# Autodesk Inventor assembly: Tamale - V1
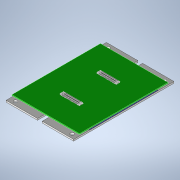
[picture p0: Inventor's stored thumbnail of the model, 180x180]
Saved by Autodesk Inventor 2022 (Build 260153000, 153)
## iProperties
Created: 2022-02-01
Part Number: Tamale - V1
Document SubType Name: Assembly
Designer: Caleb
Author: Caleb
## Documents named in this file (8)
- C:\Users\Caleb\Desktop\nebraska-silicon-lab\Hardware\ETL\modules\tamale\Tamale - V1p2.iam
- C:\Users\Caleb\Desktop\nebraska-silicon-lab\Hardware\ETL\modules\tamale\BBM.iam
- C:\Users\Caleb\Desktop\nebraska-silicon-lab\Hardware\ETL\modules\tamale\Coverplate Film.ipt
- C:\Users\Caleb\Desktop\nebraska-silicon-lab\Hardware\ETL\modules\tamale\Sensor Placement Film.ipt
- C:\Users\Caleb\Desktop\nebraska-silicon-lab\Hardware\ETL\modules\tamale\Mock Module PCB - V2p2.iam
- C:\Users\Caleb\Desktop\nebraska-silicon-lab\Hardware\ETL\modules\tamale\Long Wirebond A.ipt
- C:\Users\Caleb\Desktop\nebraska-silicon-lab\Hardware\ETL\modules\tamale\Long Wirebond B.ipt
- C:\Users\Caleb\Desktop\nebraska-silicon-lab\Hardware\ETL\modules\tamale\Baseplate Extended.ipt
## Components (150 placed, 7 different names)
1. Baseplate Extended:1 — Mate:12, Angle:5, Flush:15
2. BBM:1 [sub-assembly] — Mate:2, Angle:2, Flush:1, Flush:4, Mate:5, Flush:11
3. BBM:2 [sub-assembly] — Mate:3, Angle:1, Flush:2, Flush:4
4. BBM:3 [sub-assembly] — Mate:1, Angle:3, Flush:1, Flush:3, Mate:5, Mate:6, Flush:12
5. BBM:4 [sub-assembly] — Mate:4, Angle:4, Flush:2, Flush:3, Mate:6, Mate:10, Mate:11, Flush:9, Flush:10, Flush:14
6. Mock Module PCB - V2p2:1 [sub-assembly] — Mate:1, Mate:2, Mate:3, Mate:4, Angle:1, Angle:2, Angle:3, Angle:4, Flush:11, Angle:5, Flush:15
7. Coverplate Film:1 — Mate:10, Flush:12, Flush:14, Mate:12
8. Sensor Placement Film:1 — Mate:11, Flush:9, Flush:10
9. Long Wirebond A:1
10. Long Wirebond A:2
11. Long Wirebond A:3
12. Long Wirebond A:4
13. Long Wirebond A:5
14. Long Wirebond A:6
15. Long Wirebond A:7
16. Long Wirebond A:8
17. Long Wirebond A:9
18. Long Wirebond A:10
19. Long Wirebond A:11
20. Long Wirebond A:12
21. Long Wirebond A:13
22. Long Wirebond A:14
23. Long Wirebond A:15
24. Long Wirebond A:16
25. Long Wirebond A:17
26. Long Wirebond A:18
27. Long Wirebond A:19
28. Long Wirebond A:20
29. Long Wirebond A:21
30. Long Wirebond A:22
31. Long Wirebond A:23
32. Long Wirebond A:24
33. Long Wirebond A:25
34. Long Wirebond A:26
35. Long Wirebond A:27
36. Long Wirebond A:28
37. Long Wirebond A:29
38. Long Wirebond A:30
39. Long Wirebond A:31
40. Long Wirebond A:32
41. Long Wirebond A:33
42. Long Wirebond A:34
43. Long Wirebond A:35
44. Long Wirebond A:36
45. Long Wirebond A:37
46. Long Wirebond A:38
47. Long Wirebond A:39
48. Long Wirebond A:40
49. Long Wirebond A:41
50. Long Wirebond A:42
51. Long Wirebond A:43
52. Long Wirebond A:44
53. Long Wirebond A:45
54. Long Wirebond A:46
55. Long Wirebond A:47
56. Long Wirebond A:48
57. Long Wirebond A:49
58. Long Wirebond A:50
59. Long Wirebond A:51
60. Long Wirebond A:52
61. Long Wirebond A:53
62. Long Wirebond A:54
63. Long Wirebond A:55
64. Long Wirebond A:56
65. Long Wirebond A:57
66. Long Wirebond A:58
67. Long Wirebond A:59
68. Long Wirebond A:60
69. Long Wirebond A:61
70. Long Wirebond A:62
71. Long Wirebond A:63
72. Long Wirebond A:64
73. Long Wirebond A:65
74. Long Wirebond A:66
75. Long Wirebond A:67
76. Long Wirebond A:68
77. Long Wirebond A:69
78. Long Wirebond A:70
79. Long Wirebond A:71
80. Long Wirebond B:1
81. Long Wirebond B:2
82. Long Wirebond B:3
83. Long Wirebond B:4
84. Long Wirebond B:5
85. Long Wirebond B:6
86. Long Wirebond B:7
87. Long Wirebond B:8
88. Long Wirebond B:9
89. Long Wirebond B:10
90. Long Wirebond B:11
91. Long Wirebond B:12
92. Long Wirebond B:13
93. Long Wirebond B:14
94. Long Wirebond B:15
95. Long Wirebond B:16
96. Long Wirebond B:17
97. Long Wirebond B:18
98. Long Wirebond B:19
99. Long Wirebond B:20
100. Long Wirebond B:21
101. Long Wirebond B:22
102. Long Wirebond B:23
103. Long Wirebond B:24
104. Long Wirebond B:25
105. Long Wirebond B:26
106. Long Wirebond B:27
107. Long Wirebond B:28
108. Long Wirebond B:29
109. Long Wirebond B:30
110. Long Wirebond B:31
111. Long Wirebond B:32
112. Long Wirebond B:33
113. Long Wirebond B:34
114. Long Wirebond B:35
115. Long Wirebond B:36
116. Long Wirebond B:37
117. Long Wirebond B:38
118. Long Wirebond B:39
119. Long Wirebond B:40
120. Long Wirebond B:41
121. Long Wirebond B:42
122. Long Wirebond B:43
123. Long Wirebond B:44
124. Long Wirebond B:45
125. Long Wirebond B:46
126. Long Wirebond B:47
127. Long Wirebond B:48
128. Long Wirebond B:49
129. Long Wirebond B:50
130. Long Wirebond B:51
131. Long Wirebond B:52
132. Long Wirebond B:53
133. Long Wirebond B:54
134. Long Wirebond B:55
135. Long Wirebond B:56
136. Long Wirebond B:57
137. Long Wirebond B:58
138. Long Wirebond B:59
139. Long Wirebond B:60
140. Long Wirebond B:61
141. Long Wirebond B:62
142. Long Wirebond B:63
143. Long Wirebond B:64
144. Long Wirebond B:65
145. Long Wirebond B:66
146. Long Wirebond B:67
147. Long Wirebond B:68
148. Long Wirebond B:69
149. Long Wirebond B:70
150. Long Wirebond B:71
## Component patterns: (71 elements, first: Long Wirebond A:1), (71 elements, first: Long Wirebond B:1)
## Relationships (24: Flush 10, Mate 9, Angle 5)
- Mate:1 (0.08 mm): BBM:3 ↔ Mock Module PCB - V2p2:1
- Mate:2 (0.08 mm): BBM:1 ↔ Mock Module PCB - V2p2:1
- Mate:3 (0.08 mm): BBM:2 ↔ Mock Module PCB - V2p2:1
- Mate:4 (0.08 mm): BBM:4 ↔ Mock Module PCB - V2p2:1
- Angle:1 (0 deg): BBM:2 ↔ Mock Module PCB - V2p2:1
- Angle:2 (0 deg): BBM:1 ↔ Mock Module PCB - V2p2:1
- Angle:3 (0 deg): BBM:3 ↔ Mock Module PCB - V2p2:1
- Angle:4 (0 deg): BBM:4 ↔ Mock Module PCB - V2p2:1
- Flush:1: BBM:1 ↔ BBM:3
- Flush:2: BBM:2 ↔ BBM:4
- Flush:3: BBM:3 ↔ BBM:4
- Flush:4: BBM:1 ↔ BBM:2
- Mate:5 (0.2 mm): BBM:1 ↔ BBM:3
- Mate:6 (0.2 mm): BBM:3 ↔ BBM:4
- Mate:10: BBM:4 ↔ Coverplate Film:1
- Mate:11: BBM:4 ↔ Sensor Placement Film:1
- Flush:9: BBM:4 ↔ Sensor Placement Film:1
- Flush:10: BBM:4 ↔ Sensor Placement Film:1
- Flush:11 (0.25 mm): BBM:1 ↔ Mock Module PCB - V2p2:1
- Flush:12: BBM:3 ↔ Coverplate Film:1
- Flush:14: BBM:4 ↔ Coverplate Film:1
- Mate:12: Baseplate Extended:1 ↔ Coverplate Film:1
- Angle:5 (0 deg): Baseplate Extended:1 ↔ Mock Module PCB - V2p2:1
- Flush:15: Baseplate Extended:1 ↔ Mock Module PCB - V2p2:1
